# Autodesk Inventor assembly: AQS AssemblyRoofMount
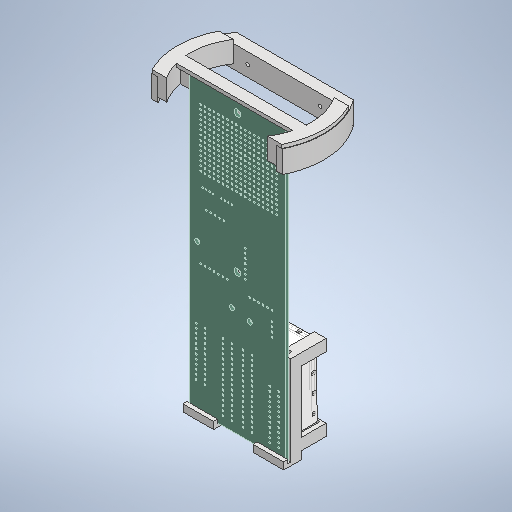
[picture p0: Inventor's stored thumbnail of the model, 512x512]
Saved by Autodesk Inventor 2025 (Build 290162010, 162A)
## iProperties
Created: 2024-07-03
Part Number: AQS AssemblyRoofMount
Document SubType Name: Assembly
Designer: vncnt
Author: vncnt
## Documents named in this file (8)
- C:\Users\vncnt\City Tech Dropbox\Vincent Ching\Community Sensor Lab Program\CAD\Air Quality Board Mount\AQS AssemblyRoofMount.iam
- C:\Users\vncnt\City Tech Dropbox\Vincent Ching\Community Sensor Lab Program\CAD\Air Quality Board Mount\PVC.ipt
- C:\Users\vncnt\City Tech Dropbox\Vincent Ching\Community Sensor Lab Program\CAD\Air Quality Board Mount\CSL_AQS_V1_spin3.iam
- C:\Users\vncnt\City Tech Dropbox\Vincent Ching\Community Sensor Lab Program\CAD\Air Quality Board Mount\AQS_Mount_V5.ipt
- C:\Users\vncnt\City Tech Dropbox\Vincent Ching\Community Sensor Lab Program\CAD\Air Quality Board Mount\SEN5X_Mount_V5.ipt
- C:\Users\vncnt\City Tech Dropbox\Vincent Ching\Community Sensor Lab Program\CAD\Air Quality Board Mount\Sensirion_STEP_SEN5x\Sensirion_STEP_SEN5x.ipt
- C:\Users\vncnt\City Tech Dropbox\Vincent Ching\Community Sensor Lab Program\CAD\Air Quality Board Mount\3in End Cap\3in End Cap.ipt
- C:\Users\vncnt\City Tech Dropbox\Vincent Ching\Community Sensor Lab Program\CAD\Air Quality Board Mount\Roof_Mount.ipt
## Components (7 placed, 7 different names)
1. PVC:1 — Flush:1, Mate:11, Flush:2, Mate:12, Mate:13
2. SEN5X_Mount_V5:1 — Mate:2, Mate:3, Mate:4, Mate:5, Mate:6, Mate:7
3. Sensirion_STEP_SEN5x:1 — Mate:4, Mate:6, Mate:7
4. CSL_AQS_V1_spin3:1 [sub-assembly] — Mate:2, Mate:3, Mate:5, Mate:14
5. 3in End Cap:1 — Flush:1, Mate:11, Flush:2
6. AQS_Mount_V5:1 — Mate:12, Mate:13, Mate:14, Mate:15, Mate:16
7. Roof_Mount:1 — Mate:15, Mate:16
## Relationships (14: Mate 12, Flush 2)
- Mate:2: SEN5X_Mount_V5:1 ↔ CSL_AQS_V1_spin3:1
- Mate:3: SEN5X_Mount_V5:1 ↔ CSL_AQS_V1_spin3:1
- Mate:4: SEN5X_Mount_V5:1 ↔ Sensirion_STEP_SEN5x:1
- Mate:5: SEN5X_Mount_V5:1 ↔ CSL_AQS_V1_spin3:1
- Mate:6: SEN5X_Mount_V5:1 ↔ Sensirion_STEP_SEN5x:1
- Mate:7: SEN5X_Mount_V5:1 ↔ Sensirion_STEP_SEN5x:1
- Flush:1: PVC:1 ↔ 3in End Cap:1
- Mate:11: PVC:1 ↔ 3in End Cap:1
- Flush:2: PVC:1 ↔ 3in End Cap:1
- Mate:12: PVC:1 ↔ AQS_Mount_V5:1
- Mate:13: PVC:1 ↔ AQS_Mount_V5:1
- Mate:14: CSL_AQS_V1_spin3:1 ↔ AQS_Mount_V5:1
- Mate:15: AQS_Mount_V5:1 ↔ Roof_Mount:1
- Mate:16: AQS_Mount_V5:1 ↔ Roof_Mount:1
